# Autodesk Inventor assembly: TS_V1_Fallmagazin_gesamt
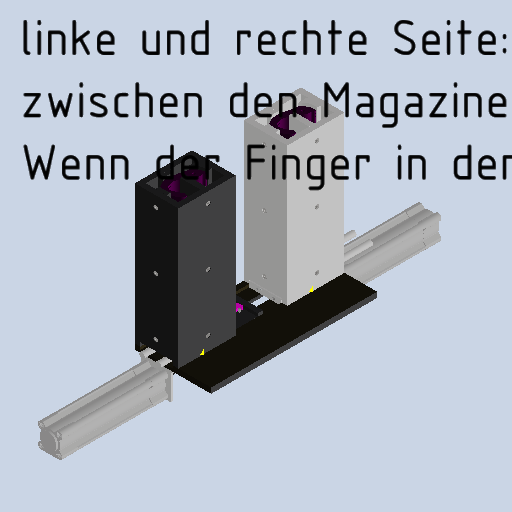
[picture p0: Inventor's stored thumbnail of the model, 512x512]
Saved by Autodesk Inventor 2025.1 (Build 291241000, 241)
## iProperties
Created: 2025-06-10
Part Number: TS_V1_Fallmagazin_gesamt
Document SubType Name: Assembly
Designer: tino
Author: tino
## Documents named in this file (17)
- C:\Users\Erik\Erik\Hochschule\3. Semester\CAD\CAD-Paspa\Useless Box\Eigene Bauteile\Fallmagazin\TS_V1_Fallmagazin_gesamt.iam
- C:\Users\Erik\Erik\Hochschule\3. Semester\CAD\CAD-Paspa\Useless Box\Eigene Bauteile\Fallmagazin\TS_V1_Fallmagazin_Boden_int.ipt
- C:\Users\Erik\Erik\Hochschule\3. Semester\CAD\CAD-Paspa\Useless Box\Eigene Bauteile\Fallmagazin\TS_V1_Fallmagazin_Wandung_int.ipt
- C:\Users\Erik\Erik\Hochschule\3. Semester\CAD\CAD-Paspa\Useless Box\Eigene Bauteile\Fallmagazin\TS_V1_Fallmagazin_Leitbleche_vorne_int.ipt
- C:\Users\Erik\Erik\Hochschule\3. Semester\CAD\CAD-Paspa\Useless Box\_Useless_Box\Finger.ipt
- C:\Users\Erik\Erik\Hochschule\3. Semester\CAD\CAD-Paspa\Useless Box\Eigene Bauteile\Fallmagazin\TS_V1_Fallmagazin_Schieber.iam
- C:\Users\Erik\Erik\Hochschule\3. Semester\CAD\CAD-Paspa\Useless Box\Kaufteile\Festo_Normzylinder_100\1376426 DSBC-32-100-PPVA-N3---(0).iam
- C:\Users\Erik\Erik\Hochschule\3. Semester\CAD\CAD-Paspa\Useless Box\Kaufteile\Festo_Normzylinder_100\1376426 DSBC-32-100-PPVA-N3---(0)_MIR.iam
- C:\Users\Erik\Erik\Hochschule\3. Semester\CAD\CAD-Paspa\Useless Box\Standart Bauteile\ISO 4762 - M4 x 12ISO.ipt
- C:\Users\Erik\Erik\Hochschule\3. Semester\CAD\CAD-Paspa\Useless Box\Standart Bauteile\ISO 4762 - M4 x 16ISO.ipt
- C:\Users\Erik\Erik\Hochschule\3. Semester\CAD\CAD-Paspa\Useless Box\Eigene Bauteile\Fallmagazin\TS_V1_Fallmagazin_Zylinderanbindung_int.ipt
- C:\Users\Erik\Erik\Hochschule\3. Semester\CAD\CAD-Paspa\Useless Box\Eigene Bauteile\Fallmagazin\TS_V1_Fallmagazin_Stopper_int.ipt
- C:\Users\Erik\Erik\Hochschule\3. Semester\CAD\CAD-Paspa\Useless Box\Eigene Bauteile\Fallmagazin\TS_V1_Fallmagazin_Zylinderhalter_int.ipt
- C:\Users\Erik\Erik\Hochschule\3. Semester\CAD\CAD-Paspa\Useless Box\Standart Bauteile\ISO 4762 - M5 x 8ISO.ipt
- C:\Users\Erik\Erik\Hochschule\3. Semester\CAD\CAD-Paspa\Useless Box\Standart Bauteile\ISO 4762 - M5 x 20ISO.ipt
- C:\Users\Erik\Erik\Hochschule\3. Semester\CAD\CAD-Paspa\Useless Box\Standart Bauteile\DIN EN ISO 2338 - 4 m6 x 10.ipt
- C:\Users\Erik\Erik\Hochschule\3. Semester\CAD\CAD-Paspa\Useless Box\Standart Bauteile\DIN 7991 - M5x12.ipt
## Components (171 placed, 16 different names)
1. TS_V1_Fallmagazin_Boden_int:1 — Mate:16, Mate:17, Mate:21, Mate:23, Mate:25, Mate:26, Mate:30, Mate:31, Mate:43, Mate:44, Mate:45, Mate:46, Mate:51, Flush:15, Mate:59, Mate:60, Flush:18, Mate:78, Mate:79, Mate:84, Mate:85, Mate:86, Mate:87, Flush:19, Flush:91
2. TS_V1_Fallmagazin_Wandung_int:2 — Mate:7, Mate:8, Flush:4, Angle:1, Angle:2, Mate:16, Mate:17, Mate:35, Mate:36, Mate:37, Mate:38, Mate:39, Mate:40, Mate:41, Mate:42, Angle:3, Flush:19
3. TS_V1_Fallmagazin_Leitbleche_vorne_int:1 — Mate:7, Mate:8, Flush:4, Tangent:2, Tangent:5, Flush:12
4. TS_V1_Fallmagazin_Schieber:1 [sub-assembly] — Mate:21, Mate:25, Mate:26, Mate:52, Mate:53, Mate:61, Mate:62, Mate:63, Mate:64, Mate:88, Tangent:6
5. TS_V1_Fallmagazin_Schieber:2 [sub-assembly] — Mate:23, Mate:30, Mate:31, Mate:56, Mate:57, Mate:65, Mate:66, Mate:67, Mate:89, Tangent:7
6. 1376426 DSBC-32-100-PPVA-N3---(0):1 [sub-assembly] — Mate:54, Mate:59, Flush:17, Flush:18, Mate:68, Mate:69, Mate:70
7. 1376426 DSBC-32-100-PPVA-N3---(0)_MIR:1 [sub-assembly] — Mate:51, Flush:15, Mate:58, Mate:60, Flush:17, Mate:75, Mate:76, Mate:77
8. TS_V1_Fallmagazin_Wandung_int:3 — Mate:45, Mate:46, Mate:47, Flush:14, Mate:48, Flush:91
9. TS_V1_Fallmagazin_Leitbleche_vorne_int:2 — Mate:47, Flush:14, Mate:48
10. TS_V1_Fallmagazin_Zylinderanbindung_int:1 — Mate:52, Mate:53, Mate:54
11. TS_V1_Fallmagazin_Zylinderanbindung_int:2 — Mate:56, Mate:57, Mate:58
12. TS_V1_Fallmagazin_Stopper_int:1 — Mate:61, Mate:62, Angle:3
13. TS_V1_Fallmagazin_Stopper_int:2 — Mate:63, Mate:64
14. TS_V1_Fallmagazin_Stopper_int:3 — Mate:65, Flush:16, Mate:67
15. TS_V1_Fallmagazin_Stopper_int:4 — Mate:66, Flush:16
16. TS_V1_Fallmagazin_Zylinderhalter_int:1 — Mate:68, Mate:69, Mate:70, Mate:71, Mate:72, Mate:73, Mate:74
17. TS_V1_Fallmagazin_Zylinderhalter_int:2 — Mate:75, Mate:76, Mate:77, Mate:78, Mate:79, Mate:80, Mate:81, Mate:82, Mate:83
18. DIN EN ISO 2338 4 m6 x 10:1 — Mate:84, Mate:85
19. DIN EN ISO 2338 4 m6 x 10:2 — Mate:86, Mate:87
20. DIN 7991 M5x12:1 — Mate:88, Tangent:6
21. DIN 7991 M5x12:2 — Mate:89, Tangent:7
22. Finger:1 — Angle:1, Tangent:2, Tangent:5, Angle:2, Flush:12
23. Finger:2
24. Finger:3
25. Finger:4
26. Finger:5
27. Finger:6
28. Finger:7
29. Finger:8
30. Finger:9
31. Finger:10
32. Finger:11
33. Finger:12
34. Finger:13
35. Finger:14
36. Finger:15
37. Finger:16
38. Finger:17
39. Finger:18
40. Finger:19
41. Finger:20
42. Finger:21
43. Finger:22
44. Finger:23
45. Finger:24
46. Finger:25
47. Finger:26
48. Finger:27
49. Finger:28
50. Finger:29
51. Finger:30
52. Finger:31
53. Finger:32
54. Finger:33
55. Finger:34
56. Finger:35
57. Finger:36
58. Finger:37
59. Finger:38
60. Finger:39
61. Finger:40
62. Finger:41
63. Finger:42
64. Finger:43
65. Finger:44
66. Finger:45
67. Finger:46
68. Finger:47
69. Finger:48
70. Finger:49
71. Finger:50
72. Finger:51
73. Finger:52
74. Finger:53
75. Finger:54
76. Finger:55
77. Finger:56
78. Finger:57
79. Finger:58
80. Finger:59
81. Finger:60
82. Finger:61
83. Finger:62
84. Finger:63
85. Finger:64
86. Finger:65
87. Finger:66
88. Finger:67
89. Finger:68
90. Finger:69
91. Finger:70
92. Finger:71
93. Finger:72
94. Finger:73
95. Finger:74
96. Finger:75
97. Finger:76
98. Finger:77
99. Finger:78
100. Finger:79
101. Finger:80
102. Finger:81
103. Finger:82
104. Finger:83
105. Finger:84
106. Finger:85
107. Finger:86
108. Finger:87
109. Finger:88
110. Finger:89
111. Finger:90
112. Finger:91
113. Finger:92
114. Finger:93
115. Finger:94
116. Finger:95
117. Finger:96
118. Finger:97
119. Finger:98
120. ISO 4762 M5 x 8:1 — Mate:71, Mate:72
121. ISO 4762 M5 x 8:2
122. ISO 4762 M5 x 8:3
123. ISO 4762 M5 x 8:4
124. ISO 4762 M5 x 20:1 — Mate:73, Mate:74
125. ISO 4762 M5 x 20:2
126. ISO 4762 M5 x 20:3
127. ISO 4762 M5 x 20:4
128. ISO 4762 M5 x 8:5 — Mate:80, Mate:81
129. ISO 4762 M5 x 8:6
130. ISO 4762 M5 x 8:7
131. ISO 4762 M5 x 8:8
132. ISO 4762 M5 x 20:5 — Mate:82, Mate:83
133. ISO 4762 M5 x 20:6
134. ISO 4762 M5 x 20:7
135. ISO 4762 M5 x 20:8
136. ISO 4762 M4 x 12:1 — Mate:35, Mate:36
137. ISO 4762 M4 x 12:2
138. ISO 4762 M4 x 12:3
139. ISO 4762 M4 x 12:4 — Mate:37, Mate:38
140. ISO 4762 M4 x 12:5
141. ISO 4762 M4 x 12:6
142. ISO 4762 M4 x 12:7 — Mate:39, Mate:40
143. ISO 4762 M4 x 12:8
144. ISO 4762 M4 x 12:9
145. ISO 4762 M4 x 12:10 — Mate:41, Mate:42
146. ISO 4762 M4 x 12:11
147. ISO 4762 M4 x 12:12
148. ISO 4762 M4 x 16:1 — Mate:43, Mate:44
149. ISO 4762 M4 x 16:2
150. ISO 4762 M4 x 16:3
151. ISO 4762 M4 x 16:4
152. ISO 4762 M4 x 16:5
153. ISO 4762 M4 x 16:6
154. ISO 4762 M4 x 12:13
155. ISO 4762 M4 x 12:14
156. ISO 4762 M4 x 12:15
157. ISO 4762 M4 x 12:16
158. ISO 4762 M4 x 12:17
159. ISO 4762 M4 x 12:18
160. ISO 4762 M4 x 12:19
161. ISO 4762 M4 x 12:20
162. ISO 4762 M4 x 12:21
163. ISO 4762 M4 x 12:22
164. ISO 4762 M4 x 12:23
165. ISO 4762 M4 x 12:24
166. ISO 4762 M4 x 16:7
167. ISO 4762 M4 x 16:8
168. ISO 4762 M4 x 16:9
169. ISO 4762 M4 x 16:10
170. ISO 4762 M4 x 16:11
171. ISO 4762 M4 x 16:12
## Component patterns: (2 elements), (98 elements, first: Finger:1), (4 elements, first: ISO 4762 M5 x 8:1), (4 elements, first: ISO 4762 M5 x 20:1), (4 elements, first: ISO 4762 M5 x 8:5), (4 elements, first: ISO 4762 M5 x 20:5), (3 elements, first: ISO 4762 M4 x 12:1), (3 elements, first: ISO 4762 M4 x 12:4), (3 elements, first: ISO 4762 M4 x 12:7), (3 elements, first: ISO 4762 M4 x 12:10), (6 elements, first: ISO 4762 M4 x 16:1), Komponentenanordnung 2:2 (3 elements), Komponentenanordnung 3:2 (3 elements), Komponentenanordnung 4:2 (3 elements), Komponentenanordnung 5:2 (3 elements), Komponentenanordnung 6:2 (6 elements)
## Relationships (78: Mate 62, Flush 9, Tangent 4, Angle 3)
- Mate:7: TS_V1_Fallmagazin_Wandung_int:2 ↔ TS_V1_Fallmagazin_Leitbleche_vorne_int:1
- Mate:8: TS_V1_Fallmagazin_Wandung_int:2 ↔ TS_V1_Fallmagazin_Leitbleche_vorne_int:1
- Flush:4: TS_V1_Fallmagazin_Wandung_int:2 ↔ TS_V1_Fallmagazin_Leitbleche_vorne_int:1
- Angle:1 (0 deg): TS_V1_Fallmagazin_Wandung_int:2 ↔ Finger:1
- Tangent:2: TS_V1_Fallmagazin_Leitbleche_vorne_int:1 ↔ Finger:1
- Tangent:5: TS_V1_Fallmagazin_Leitbleche_vorne_int:1 ↔ Finger:1
- Angle:2 (0 deg): TS_V1_Fallmagazin_Wandung_int:2 ↔ Finger:1
- Mate:16: TS_V1_Fallmagazin_Boden_int:1 ↔ TS_V1_Fallmagazin_Wandung_int:2
- Mate:17: TS_V1_Fallmagazin_Boden_int:1 ↔ TS_V1_Fallmagazin_Wandung_int:2
- Mate:21: TS_V1_Fallmagazin_Boden_int:1 ↔ TS_V1_Fallmagazin_Schieber:1
- Mate:23: TS_V1_Fallmagazin_Boden_int:1 ↔ TS_V1_Fallmagazin_Schieber:2
- Mate:25: TS_V1_Fallmagazin_Boden_int:1 ↔ TS_V1_Fallmagazin_Schieber:1
- Mate:26: TS_V1_Fallmagazin_Boden_int:1 ↔ TS_V1_Fallmagazin_Schieber:1
- Mate:30: TS_V1_Fallmagazin_Boden_int:1 ↔ TS_V1_Fallmagazin_Schieber:2
- Mate:31: TS_V1_Fallmagazin_Boden_int:1 ↔ TS_V1_Fallmagazin_Schieber:2
- Mate:35: TS_V1_Fallmagazin_Wandung_int:2 ↔ ISO 4762 M4 x 12:1
- Mate:36: TS_V1_Fallmagazin_Wandung_int:2 ↔ ISO 4762 M4 x 12:1
- Mate:37: TS_V1_Fallmagazin_Wandung_int:2 ↔ ISO 4762 M4 x 12:4
- Mate:38: TS_V1_Fallmagazin_Wandung_int:2 ↔ ISO 4762 M4 x 12:4
- Mate:39: TS_V1_Fallmagazin_Wandung_int:2 ↔ ISO 4762 M4 x 12:7
- Mate:40: TS_V1_Fallmagazin_Wandung_int:2 ↔ ISO 4762 M4 x 12:7
- Mate:41: TS_V1_Fallmagazin_Wandung_int:2 ↔ ISO 4762 M4 x 12:10
- Mate:42: TS_V1_Fallmagazin_Wandung_int:2 ↔ ISO 4762 M4 x 12:10
- Mate:43: TS_V1_Fallmagazin_Boden_int:1 ↔ ISO 4762 M4 x 16:1
- Mate:44: TS_V1_Fallmagazin_Boden_int:1 ↔ ISO 4762 M4 x 16:1
- Flush:12: TS_V1_Fallmagazin_Leitbleche_vorne_int:1 ↔ Finger:1
- Mate:45: TS_V1_Fallmagazin_Boden_int:1 ↔ TS_V1_Fallmagazin_Wandung_int:3
- Mate:46: TS_V1_Fallmagazin_Boden_int:1 ↔ TS_V1_Fallmagazin_Wandung_int:3
- Mate:47: TS_V1_Fallmagazin_Wandung_int:3 ↔ TS_V1_Fallmagazin_Leitbleche_vorne_int:2
- Flush:14: TS_V1_Fallmagazin_Wandung_int:3 ↔ TS_V1_Fallmagazin_Leitbleche_vorne_int:2
- Mate:48: TS_V1_Fallmagazin_Wandung_int:3 ↔ TS_V1_Fallmagazin_Leitbleche_vorne_int:2
- Mate:51 (4 mm): TS_V1_Fallmagazin_Boden_int:1 ↔ 1376426 DSBC-32-100-PPVA-N3---(0)_MIR:1
- Flush:15: TS_V1_Fallmagazin_Boden_int:1 ↔ 1376426 DSBC-32-100-PPVA-N3---(0)_MIR:1
- Mate:52: TS_V1_Fallmagazin_Schieber:1 ↔ TS_V1_Fallmagazin_Zylinderanbindung_int:1
- Mate:53: TS_V1_Fallmagazin_Schieber:1 ↔ TS_V1_Fallmagazin_Zylinderanbindung_int:1
- Mate:54: 1376426 DSBC-32-100-PPVA-N3---(0):1 ↔ TS_V1_Fallmagazin_Zylinderanbindung_int:1
- Mate:56: TS_V1_Fallmagazin_Schieber:2 ↔ TS_V1_Fallmagazin_Zylinderanbindung_int:2
- Mate:57: TS_V1_Fallmagazin_Schieber:2 ↔ TS_V1_Fallmagazin_Zylinderanbindung_int:2
- Mate:58: 1376426 DSBC-32-100-PPVA-N3---(0)_MIR:1 ↔ TS_V1_Fallmagazin_Zylinderanbindung_int:2
- Mate:59 (-16.4 mm): TS_V1_Fallmagazin_Boden_int:1 ↔ 1376426 DSBC-32-100-PPVA-N3---(0):1
- Mate:60 (-16.4 mm): TS_V1_Fallmagazin_Boden_int:1 ↔ 1376426 DSBC-32-100-PPVA-N3---(0)_MIR:1
- Mate:61: TS_V1_Fallmagazin_Schieber:1 ↔ TS_V1_Fallmagazin_Stopper_int:1
- Mate:62: TS_V1_Fallmagazin_Schieber:1 ↔ TS_V1_Fallmagazin_Stopper_int:1
- Mate:63: TS_V1_Fallmagazin_Schieber:1 ↔ TS_V1_Fallmagazin_Stopper_int:2
- Mate:64: TS_V1_Fallmagazin_Schieber:1 ↔ TS_V1_Fallmagazin_Stopper_int:2
- Mate:65: TS_V1_Fallmagazin_Schieber:2 ↔ TS_V1_Fallmagazin_Stopper_int:3
- Mate:66: TS_V1_Fallmagazin_Schieber:2 ↔ TS_V1_Fallmagazin_Stopper_int:4
- Flush:16: TS_V1_Fallmagazin_Stopper_int:3 ↔ TS_V1_Fallmagazin_Stopper_int:4
- Mate:67: TS_V1_Fallmagazin_Schieber:2 ↔ TS_V1_Fallmagazin_Stopper_int:3
- Flush:17: 1376426 DSBC-32-100-PPVA-N3---(0):1 ↔ 1376426 DSBC-32-100-PPVA-N3---(0)_MIR:1
- Flush:18: TS_V1_Fallmagazin_Boden_int:1 ↔ 1376426 DSBC-32-100-PPVA-N3---(0):1
- Mate:68: 1376426 DSBC-32-100-PPVA-N3---(0):1 ↔ TS_V1_Fallmagazin_Zylinderhalter_int:1
- Mate:69: 1376426 DSBC-32-100-PPVA-N3---(0):1 ↔ TS_V1_Fallmagazin_Zylinderhalter_int:1
- Mate:70: 1376426 DSBC-32-100-PPVA-N3---(0):1 ↔ TS_V1_Fallmagazin_Zylinderhalter_int:1
- Mate:71: TS_V1_Fallmagazin_Zylinderhalter_int:1 ↔ ISO 4762 M5 x 8:1
- Mate:72: TS_V1_Fallmagazin_Zylinderhalter_int:1 ↔ ISO 4762 M5 x 8:1
- Mate:73: TS_V1_Fallmagazin_Zylinderhalter_int:1 ↔ ISO 4762 M5 x 20:1
- Mate:74: TS_V1_Fallmagazin_Zylinderhalter_int:1 ↔ ISO 4762 M5 x 20:1
- Mate:75: 1376426 DSBC-32-100-PPVA-N3---(0)_MIR:1 ↔ TS_V1_Fallmagazin_Zylinderhalter_int:2
- Mate:76: 1376426 DSBC-32-100-PPVA-N3---(0)_MIR:1 ↔ TS_V1_Fallmagazin_Zylinderhalter_int:2
- Mate:77: 1376426 DSBC-32-100-PPVA-N3---(0)_MIR:1 ↔ TS_V1_Fallmagazin_Zylinderhalter_int:2
- Mate:78: TS_V1_Fallmagazin_Boden_int:1 ↔ TS_V1_Fallmagazin_Zylinderhalter_int:2
- Mate:79: TS_V1_Fallmagazin_Boden_int:1 ↔ TS_V1_Fallmagazin_Zylinderhalter_int:2
- Mate:80: TS_V1_Fallmagazin_Zylinderhalter_int:2 ↔ ISO 4762 M5 x 8:5
- Mate:81: TS_V1_Fallmagazin_Zylinderhalter_int:2 ↔ ISO 4762 M5 x 8:5
- Mate:82: TS_V1_Fallmagazin_Zylinderhalter_int:2 ↔ ISO 4762 M5 x 20:5
- Mate:83: TS_V1_Fallmagazin_Zylinderhalter_int:2 ↔ ISO 4762 M5 x 20:5
- Mate:84: TS_V1_Fallmagazin_Boden_int:1 ↔ DIN EN ISO 2338 4 m6 x 10:1
- Mate:85 (0.5 mm): TS_V1_Fallmagazin_Boden_int:1 ↔ DIN EN ISO 2338 4 m6 x 10:1
- Mate:86: TS_V1_Fallmagazin_Boden_int:1 ↔ DIN EN ISO 2338 4 m6 x 10:2
- Mate:87 (1 mm): TS_V1_Fallmagazin_Boden_int:1 ↔ DIN EN ISO 2338 4 m6 x 10:2
- Angle:3 (0 deg): TS_V1_Fallmagazin_Wandung_int:2 ↔ TS_V1_Fallmagazin_Stopper_int:1
- Mate:88: TS_V1_Fallmagazin_Schieber:1 ↔ DIN 7991 M5x12:1
- Tangent:6: TS_V1_Fallmagazin_Schieber:1 ↔ DIN 7991 M5x12:1
- Mate:89: TS_V1_Fallmagazin_Schieber:2 ↔ DIN 7991 M5x12:2
- Tangent:7: TS_V1_Fallmagazin_Schieber:2 ↔ DIN 7991 M5x12:2
- Flush:19: TS_V1_Fallmagazin_Boden_int:1 ↔ TS_V1_Fallmagazin_Wandung_int:2
- Flush:91: TS_V1_Fallmagazin_Boden_int:1 ↔ TS_V1_Fallmagazin_Wandung_int:3
## Named parameters: Magazin_Hoehe = 255 mm, Abstand_Schrauben_vert = 105 mm, Abstand_Rand = 45 mm, Anbindung_Zylinder = 16.4 mm
